# Autodesk Inventor assembly: montagem
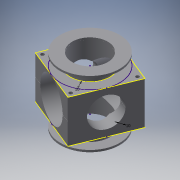
[picture p0: Inventor's stored thumbnail of the model, 180x180]
Saved by Autodesk Inventor 2019 (Build 230136000, 136)
## iProperties
Created: 2019-04-16
Part Number: montagem
Document SubType Name: Assembly
Designer: Vladimir
Author: Vladimir
## Documents named in this file (3)
- D:\GDrive\Unicamp-Mestrado\Topicos fisica exp\peca da bobina\montagem.iam
- D:\GDrive\Unicamp-Mestrado\Topicos fisica exp\peca da bobina\peca1.ipt
- D:\GDrive\Unicamp-Mestrado\Topicos fisica exp\peca da bobina\peca2.ipt
## Components (4 placed, 2 different names)
1. peca1:1 — Insert:1
2. peca2:1 — Insert:1, Insert:2, Insert:3
3. peca1:2 — Insert:4
4. peca2:2 — Insert:2, Insert:3, Insert:4
## Relationships (4: Insert 4)
- Insert:1: peca1:1 ↔ peca2:1
- Insert:2: peca2:1 ↔ peca2:2
- Insert:3: peca2:1 ↔ peca2:2
- Insert:4: peca1:2 ↔ peca2:2
